# Autodesk Inventor assembly: NP18-12
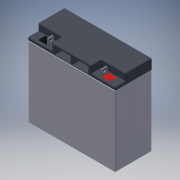
[picture p0: Inventor's stored thumbnail of the model, 180x180]
Saved by Autodesk Inventor 2016 (Build 200138000, 138)
## iProperties
Category: Controls
Company: Autodesk Inc.
Created: 2015-11-23
Part Number: NP18-12
Document SubType Name: Assembly
Designer: Autodesk Inc.
Description: Battery, ,12 volt, 18 AH, Non-spillable
Catalog Web Link: http://www.enersys.com/Genesis_NP_Batteries.aspx?langType=1033
Vendor: EnerSys
Author: Autodesk Inc.
Keywords: FIRSTChoice
## Documents named in this file (3)
- E:\1073CAD\Robot2017\DriveTrain\Belly pan with electronics\FRC KOP 2016\Electrical\fc16-036_Battery.iam
- E:\1073CAD\Robot2017\DriveTrain\Belly pan with electronics\FRC KOP 2016\Electrical\Parts\fc16-036_Top.ipt
- E:\1073CAD\Robot2017\DriveTrain\Belly pan with electronics\FRC KOP 2016\Electrical\Parts\fc16-036_Middle.ipt
## Components (2 placed, 2 different names)
1. fc16-036_Top:1 — Flush:1
2. fc16-036_Middle:1 — Flush:1, Flush:2
## Relationships (2: Flush 2)
- Flush:1: fc16-036_Top:1 ↔ fc16-036_Middle:1
- Flush:2 (-89.662 mm): fc16-036_Middle:1
